# Autodesk Inventor assembly: Mbot
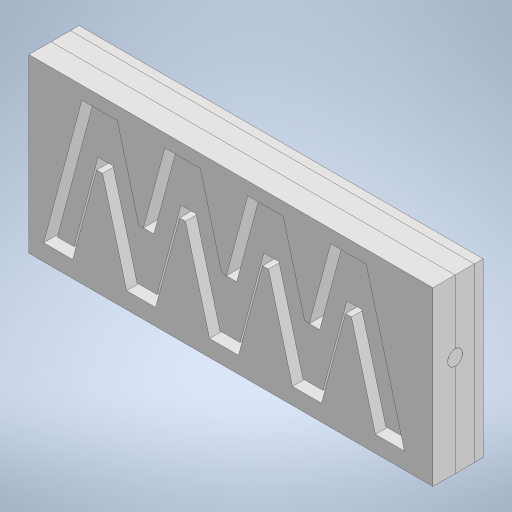
[picture p0: Inventor's stored thumbnail of the model, 512x512]
Saved by Autodesk Inventor 2024 (Build 280153000, 153)
## iProperties
Created: 2024-02-12
Part Number: Mbot
Document SubType Name: Assembly
Designer: juanp
Author: juanp
## Documents named in this file (5)
- C:\Users\juanp\Desktop\SoftRobotics\Pruebas\Fabricacion\Mbot.iam
- C:\Users\juanp\Desktop\SoftRobotics\Pruebas\Fabricacion\Solid6.ipt
- C:\Users\juanp\Desktop\SoftRobotics\Pruebas\Fabricacion\Solid7.ipt
- C:\Users\juanp\Desktop\SoftRobotics\Pruebas\Fabricacion\Solid9.ipt
- C:\Users\juanp\Desktop\SoftRobotics\Pruebas\Fabricacion\Solid10.ipt
## Components (4 placed, 4 different names)
1. Solid6:1 — Flush:2, Mate:2
2. Solid7:1 — Flush:3, Flush:5, Mate:3
3. Solid9:1 — Flush:1, Flush:2, Flush:3, Flush:4, Flush:5, Mate:1, Mate:2, Mate:3
4. Solid10:1 — Flush:1, Flush:4, Mate:1
## Relationships (8: Flush 5, Mate 3)
- Flush:1: Solid9:1 ↔ Solid10:1
- Flush:2: Solid6:1 ↔ Solid9:1
- Flush:3: Solid7:1 ↔ Solid9:1
- Flush:4: Solid9:1 ↔ Solid10:1
- Flush:5: Solid7:1 ↔ Solid9:1
- Mate:1: Solid9:1 ↔ Solid10:1
- Mate:2: Solid6:1 ↔ Solid9:1
- Mate:3: Solid7:1 ↔ Solid9:1
